# Autodesk Inventor assembly: OUTER_GEAR_HGB
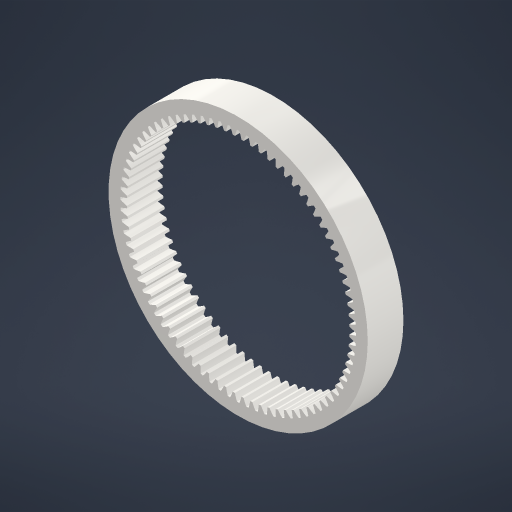
[picture p0: Inventor's stored thumbnail of the model, 512x512]
Saved by Autodesk Inventor 2024.2 (Build 282272000, 272)
## iProperties
Created: 2026-01-16
Part Number: OUTER_GEAR_HGB
Document SubType Name: Assembly
Designer: 4aida
Author: 4aida
## Documents named in this file (3)
- C:\Users\4aida\OneDrive\Documents\CADING\DESIGN FILES\STANDARDS\Harmonic_GB\OUTER_GEAR_HGB.iam
- C:\Users\4aida\OneDrive\Documents\CADING\DESIGN FILES\STANDARDS\Harmonic_GB\OUTER_GEAR_HGB\Design Accelerator\Spur Gears1.iam
- C:\Users\4aida\OneDrive\Documents\CADING\DESIGN FILES\STANDARDS\Harmonic_GB\HARMONIC_GB.xlsx
## Components (1 placed, 1 different names)
1. Spur Gears:1 [sub-assembly]
## Named parameters: N_ = 80, DP_ = 0.8 mm, OD_ = 60 mm, t_ = 3 mm, h_ = 30 mm, f_ = 5 mm
